# Autodesk Inventor assembly: servo_handle
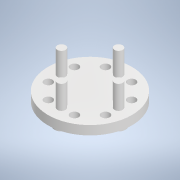
[picture p0: Inventor's stored thumbnail of the model, 180x180]
Saved by Autodesk Inventor 2021.4 (Build 254397000, 397)
## iProperties
Created: 2022-08-02
Part Number: servo_handle
Document SubType Name: Assembly
Designer: isamu
Author: isamu
## Documents named in this file (3)
- D:\personal_projects\robot\inventor\2021_matlab_compat _v2\servo_frames\servo_handle.iam
- D:\personal_projects\robot\exports\handle\servo handle 4.ipt
- D:\personal_projects\robot\exports\screws\m2x8.ipt
## Components (5 placed, 2 different names)
1. servo handle 4:1 — Insert:1, Insert:2, Insert:3, Insert:4
2. m2x8:1 — Insert:3
3. m2x8:2 — Insert:4
4. m2x8:3 — Insert:2
5. m2x8:4 — Insert:1
## Relationships (4: Insert 4)
- Insert:1: servo handle 4:1 ↔ m2x8:4
- Insert:2: servo handle 4:1 ↔ m2x8:3
- Insert:3: servo handle 4:1 ↔ m2x8:1
- Insert:4: servo handle 4:1 ↔ m2x8:2
